# Autodesk Inventor assembly: zlozenie_baza
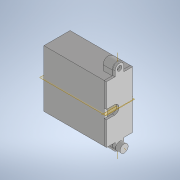
[picture p0: Inventor's stored thumbnail of the model, 180x180]
Saved by Autodesk Inventor 2021 (Build 250183000, 183)
## iProperties
Created: 2025-11-29
Part Number: zlozenie_baza
Document SubType Name: Assembly
Designer: huber
Author: huber
## Documents named in this file (4)
- C:\Users\huber\OneDrive\Pulpit\hackaton BHL\BHL 2025\zlozenie_baza.iam
- C:\Users\huber\OneDrive\Pulpit\hackaton BHL\BHL 2025\pokrywa_baza.ipt
- C:\Users\huber\OneDrive\Pulpit\hackaton BHL\BHL 2025\pudelko_baza.ipt
- C:\Users\huber\OneDrive\Pulpit\hackaton BHL\BHL 2025\sruba- m4x12.ipt
## Components (3 placed, 3 different names)
1. pokrywa_baza:1 — Insert:1, Insert:2, Insert:3
2. pudelko_baza:1 — Insert:1, Insert:2
3. sruba- m4x12:1 — Insert:3
## Relationships (3: Insert 3)
- Insert:1: pokrywa_baza:1 ↔ pudelko_baza:1
- Insert:2: pokrywa_baza:1 ↔ pudelko_baza:1
- Insert:3: pokrywa_baza:1 ↔ sruba- m4x12:1
